# Autodesk Inventor assembly: XEndBushingLeft
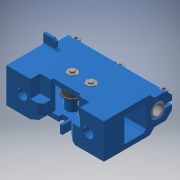
[picture p0: Inventor's stored thumbnail of the model, 180x180]
Saved by Autodesk Inventor 2016 (Build 200138000, 138)
## iProperties
Created: 2014-08-16
Part Number: XEndBushingLeft
Document SubType Name: Assembly
Designer: Jack
Mass: 125.221 g
Surface Area: 373.198 cm^2
Volume: 71.1283 cm^3
Density: 1.76049 g/cm^3
Author: Jack
Title: X End Left
## Documents named in this file (13)
- C:\Users\Jack\ownCloud\Projects\CrossBot\InventorModel\XAxis\XEndBushingLeft.iam
- C:\Users\Jack\ownCloud\Projects\CrossBot\InventorModel\Hardware\Nuts\Nut3.ipt
- C:\Users\Jack\ownCloud\Projects\CrossBot\InventorModel\Hardware\Bolts\SHCS\SHCS4\SHCS4x30.ipt
- C:\Users\Jack\ownCloud\Projects\CrossBot\InventorModel\Hardware\Nuts\Nut4.ipt
- C:\Users\Jack\ownCloud\Projects\CrossBot\InventorModel\Hardware\Bearing\BearingRadialBall\BearingRadialBallF624zz.ipt
- C:\Users\Jack\ownCloud\Projects\CrossBot\InventorModel\Hardware\Wahsers\M4Washer.ipt
- C:\Users\Jack\ownCloud\Projects\CrossBot\InventorModel\Hardware\Bolts\SHCS\SHCS3\SHCS3x8.ipt
- C:\Users\Jack\ownCloud\Projects\CrossBot\InventorModel\XAxis\XAxisBearingSpacer.ipt
- C:\Users\Jack\ownCloud\Projects\CrossBot\InventorModel\Hardware\Belt\GT2Idler.iam
- C:\Users\Jack\ownCloud\Projects\CrossBot\InventorModel\XAxis\XAxisBeltIdlerSpacer.ipt
- C:\Users\Jack\ownCloud\Projects\CrossBot\InventorModel\Hardware\Bolts\SHCS\SHCS3\SHCS3x14.ipt
- C:\Users\Jack\ownCloud\Projects\CrossBot\InventorModel\XAxis\XEndBushingLeft.ipt
- C:\Users\Jack\ownCloud\Projects\CrossBot\InventorModel\Hardware\Bearing\BearingLinear\BearingLinearPlastic\BearingPlastic8x12x12.ipt
## Components (26 placed, 12 different names)
1. XAxisBearingSpacer:2 — Mate:51, Mate:52
2. GT2Idler:1 [sub-assembly] — Mate:58, Mate:101, Mate:114
3. XAxisBeltIdlerSpacer:1 — Mate:61, Mate:76
4. XEndBushingLeft:1 — Mate:102, Mate:103, Mate:104, Angle:1, Angle:2, Angle:3, Mate:105, Mate:106, Mate:107, Mate:108, Mate:109, Angle:4, Angle:5, Mate:110, Mate:111, Mate:112, Mate:113, Mate:115, Mate:116, Angle:6, Angle:7, Mate:117, Mate:118, Mate:119, Mate:120, Flush:8, Flush:9
5. BearingPlastic8x12x12:1 — Mate:119, Flush:9
6. BearingPlastic8x12x12:2 — Mate:120, Flush:8
7. BearingRadialBallF624zz:3
8. BearingRadialBallF624zz:4
9. M4Washer:4 — Mate:38, Mate:52
10. M4Washer:3 — Mate:115
11. M4Washer:2 — Mate:30, Mate:114, Mate:116
12. M4Washer:1 — Mate:57, Mate:76, Mate:101
13. Nut4:2 — Mate:21, Angle:6, Mate:117
14. Nut4:1 — Mate:20, Angle:7, Mate:118
15. SHCS4x30:2 — Mate:20, Mate:38, Mate:51, Mate:112
16. SHCS4x30:1 — Mate:21, Mate:30, Mate:57, Mate:58, Mate:61, Mate:113
17. Nut3:3 — Mate:43, Flush:7, Angle:4, Mate:111
18. Nut3:4 — Mate:42, Flush:6, Angle:5, Mate:110
19. SHCS3x8:1 — Mate:42, Flush:6, Mate:108
20. SHCS3x8:2 — Mate:43, Flush:7, Mate:109
21. SHCS3x14:2 — Mate:92, Mate:104
22. SHCS3x14:3 — Mate:103
23. Nut3:5 — Angle:2, Mate:106
24. SHCS3x14:1 — Mate:91, Mate:102
25. Nut3:2 — Mate:92, Angle:1, Mate:107
26. Nut3:1 — Mate:91, Angle:3, Mate:105
## Relationships (52: Mate 41, Angle 7, Flush 4)
- Mate:20: Nut4:1 ↔ SHCS4x30:2
- Mate:21: Nut4:2 ↔ SHCS4x30:1
- Mate:30: M4Washer:2 ↔ SHCS4x30:1
- [Mate]: BearingRadialBallF624zz:3 ↔ BearingRadialBallF624zz:4
- [Mate]: BearingRadialBallF624zz:3 ↔ BearingRadialBallF624zz:4
- [Mate]: BearingRadialBallF624zz:3 ↔ M4Washer:3
- [Mate]: BearingRadialBallF624zz:3 ↔ M4Washer:3
- [Mate]: BearingRadialBallF624zz:4 ↔ M4Washer:4
- [Mate]: BearingRadialBallF624zz:4 ↔ M4Washer:4
- Mate:38: M4Washer:4 ↔ SHCS4x30:2
- Mate:42: Nut3:4 ↔ SHCS3x8:1
- Mate:43: Nut3:3 ↔ SHCS3x8:2
- Mate:51: XAxisBearingSpacer:2 ↔ SHCS4x30:2
- Mate:52: XAxisBearingSpacer:2 ↔ M4Washer:4
- Mate:57: M4Washer:1 ↔ SHCS4x30:1
- Mate:58: GT2Idler:1 ↔ SHCS4x30:1
- Mate:61: XAxisBeltIdlerSpacer:1 ↔ SHCS4x30:1
- Mate:76: XAxisBeltIdlerSpacer:1 ↔ M4Washer:1
- Flush:6 (-0.5 mm): Nut3:4 ↔ SHCS3x8:1
- Flush:7 (-0.5 mm): Nut3:3 ↔ SHCS3x8:2
- Mate:91: SHCS3x14:1 ↔ Nut3:1
- Mate:92: SHCS3x14:2 ↔ Nut3:2
- [Mate]: SHCS3x14:3 ↔ Nut3:5
- Mate:101: GT2Idler:1 ↔ M4Washer:1
- Mate:102: XEndBushingLeft:1 ↔ SHCS3x14:1
- Mate:103: XEndBushingLeft:1 ↔ SHCS3x14:3
- Mate:104: XEndBushingLeft:1 ↔ SHCS3x14:2
- Angle:1 (0 deg): XEndBushingLeft:1 ↔ Nut3:2
- Angle:2 (0 deg): XEndBushingLeft:1 ↔ Nut3:5
- Angle:3 (0 deg): XEndBushingLeft:1 ↔ Nut3:1
- Mate:105: XEndBushingLeft:1 ↔ Nut3:1
- Mate:106: XEndBushingLeft:1 ↔ Nut3:5
- Mate:107: XEndBushingLeft:1 ↔ Nut3:2
- Mate:108: XEndBushingLeft:1 ↔ SHCS3x8:1
- Mate:109: XEndBushingLeft:1 ↔ SHCS3x8:2
- Angle:4 (0 deg): XEndBushingLeft:1 ↔ Nut3:3
- Angle:5 (0 deg): XEndBushingLeft:1 ↔ Nut3:4
- Mate:110: XEndBushingLeft:1 ↔ Nut3:4
- Mate:111: XEndBushingLeft:1 ↔ Nut3:3
- Mate:112: XEndBushingLeft:1 ↔ SHCS4x30:2
- Mate:113: XEndBushingLeft:1 ↔ SHCS4x30:1
- Mate:114: GT2Idler:1 ↔ M4Washer:2
- Mate:115: XEndBushingLeft:1 ↔ M4Washer:3
- Mate:116: XEndBushingLeft:1 ↔ M4Washer:2
- Angle:6 (0 deg): XEndBushingLeft:1 ↔ Nut4:2
- Angle:7 (0 deg): XEndBushingLeft:1 ↔ Nut4:1
- Mate:117: XEndBushingLeft:1 ↔ Nut4:2
- Mate:118: XEndBushingLeft:1 ↔ Nut4:1
- Mate:119: XEndBushingLeft:1 ↔ BearingPlastic8x12x12:1
- Mate:120: XEndBushingLeft:1 ↔ BearingPlastic8x12x12:2
- Flush:8: XEndBushingLeft:1 ↔ BearingPlastic8x12x12:2
- Flush:9: XEndBushingLeft:1 ↔ BearingPlastic8x12x12:1
## Named parameters: d35_d44 = 0 mm, d36_d45 = 0 mm, d37_d46 = 0 mm, d38_d47 = 0 mm, d39_d48 = 0 mm, d40_d49 = 0 mm, d156_d150 = 0 mm
